# Autodesk Inventor assembly: Config PSU
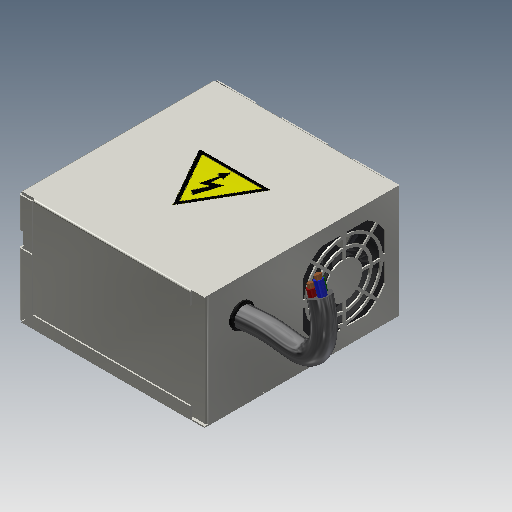
[picture p0: Inventor's stored thumbnail of the model, 512x512]
Saved by Autodesk Inventor 2020 (Build 240152000, 152)
## iProperties
Created: 2005-12-21
Part Number: Config PSU
Document SubType Name: Assembly
Designer: Simon.Ng@autodesk.com
Stock Number: NA
Description: Power Supply
Mass: 171.379 g
Surface Area: 2491.15 cm^2
Volume: 171.379 cm^3
Density: 1 g/cm^3
Company: Autodesk Asia Pte. Ltd.
Title: Purchased Part
Author: Simon.Ng@autodesk.com
Revision Number: A
## Documents named in this file (6)
- C:\Users\hallc\Desktop\Process Equipment\Workspace\Supplier Content\Electrical Design\Power Supply\Power Supply.iam
- C:\Users\hallc\Desktop\Process Equipment\Workspace\Supplier Content\Electrical Design\Power Supply\Back Casing.ipt
- C:\Users\hallc\Desktop\Process Equipment\Workspace\Supplier Content\Electrical Design\Power Supply\Top Casing.ipt
- C:\Users\hallc\Desktop\Process Equipment\Workspace\Supplier Content\Electrical Design\Power Supply\Fan.ipt
- C:\Users\hallc\Desktop\Process Equipment\Workspace\Supplier Content\Electrical Design\Power Supply\Power Supply PCB.ipt
- C:\Users\hallc\Desktop\Process Equipment\Workspace\Supplier Content\Electrical Design\Power Supply\Power Lead.ipt
## Components (5 placed, 5 different names)
1. Back Casing:1 — Mate:1, Insert:1, Angle:1, Mate:4, Mate:5, Mate:6, Flush:1
2. Top Casing:1 — Mate:4, Mate:5, Mate:6, Mate:7, Mate:8, Mate:9
3. Fan:1 — Insert:1, Angle:1
4. Power Supply PCB:1 — Mate:7, Mate:8, Mate:9
5. Power Lead:1 — Flush:1
## Relationships (10: Mate 7, Insert 1, Angle 1, Flush 1)
- Mate:1: Back Casing:1
- Insert:1: Back Casing:1 ↔ Fan:1
- Angle:1 (0 deg): Back Casing:1 ↔ Fan:1
- Mate:4: Back Casing:1 ↔ Top Casing:1
- Mate:5: Back Casing:1 ↔ Top Casing:1
- Mate:6: Back Casing:1 ↔ Top Casing:1
- Mate:7 (3.175 mm): Top Casing:1 ↔ Power Supply PCB:1
- Mate:8 (2.54 mm): Top Casing:1 ↔ Power Supply PCB:1
- Mate:9 (2.54 mm): Top Casing:1 ↔ Power Supply PCB:1
- Flush:1: Back Casing:1 ↔ Power Lead:1
